# Autodesk Inventor assembly: Z Mount
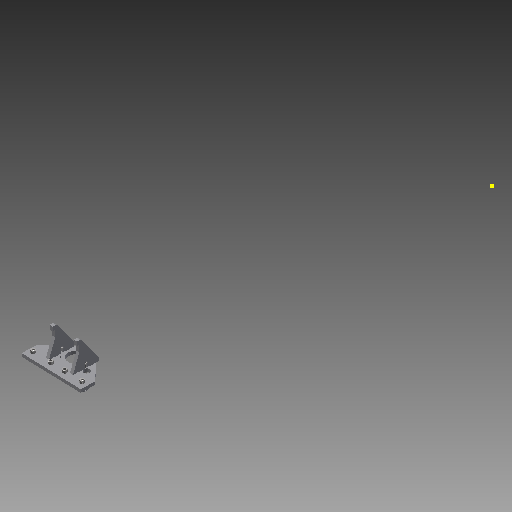
[picture p0: Inventor's stored thumbnail of the model, 512x512]
Saved by Autodesk Inventor 2017 (Build 210142000, 142)
## iProperties
Created: 2016-07-25
Part Number: Z Mount
Document SubType Name: Assembly
Designer: User
Author: User
## Documents named in this file (11)
- C:\All INVENTOR\SL-Inventor\SL-Beast 3D Printer\Z Mount.iam
- C:\All INVENTOR\SL-Inventor\SL-Beast 3D Printer\Rear Z Motor Mount.ipt
- C:\All INVENTOR\SL-Inventor\SL-Beast 3D Printer\Z Motor Mount Brace.ipt
- C:\All INVENTOR\SL-Inventor\SL-Beast 3D Printer\Z Motor Mount Brace_CPY.ipt
- C:\All INVENTOR\SL-Inventor\SL-Beast 3D Printer\en-US\ANSI B18.3.1M(6)\ANSI B18.3.1M - M3x0.5 x 16(1).ipt
- C:\All INVENTOR\SL-Inventor\SL-Beast 3D Printer\en-US\CSN EN 24 036\CSN EN 24 036 - M3.ipt
- C:\All INVENTOR\SL-Inventor\SL-Beast 3D Printer\en-US\ANSI B18.3.1M(6)\ANSI B18.3.1M - M5x0.8 x 12(1).ipt
- C:\All INVENTOR\SL-Inventor\SL-Beast 3D Printer\M5 Tee Nut-Generic_MIR1.ipt
- C:\All INVENTOR\SL-Inventor\SL-Beast 3D Printer\M5 Tee Nut-Generic_MIR1_CPY.ipt
- C:\All INVENTOR\SL-Inventor\SL-Beast 3D Printer\M5 Tee Nut-Generic_MIR1_CPY_CPY.ipt
- C:\All INVENTOR\SL-Inventor\SL-Beast 3D Printer\M5 Tee Nut-Generic_MIR1_CPY_CPY_CPY.ipt
## Components (15 placed, 10 different names)
1. Rear Z Motor Mount:1
2. Z Motor Mount Brace:1
3. Z Motor Mount Brace_CPY:1
4. Forged Socket Head Cap Screw - Metric M3x0.5 x 16:1
5. Forged Socket Head Cap Screw - Metric M3x0.5 x 16:2
6. CSN EN 24036 M3:1
7. CSN EN 24036 M3:2
8. Forged Socket Head Cap Screw - Metric M5x0.8 x 12:1
9. Forged Socket Head Cap Screw - Metric M5x0.8 x 12:2
10. Forged Socket Head Cap Screw - Metric M5x0.8 x 12:3
11. Forged Socket Head Cap Screw - Metric M5x0.8 x 12:4
12. M5 Tee Nut-Generic_MIR1:1
13. M5 Tee Nut-Generic_MIR1_CPY:1
14. M5 Tee Nut-Generic_MIR1_CPY_CPY:1
15. M5 Tee Nut-Generic_MIR1_CPY_CPY_CPY:1
## Relationships (24: Mate 14, Insert 6, Flush 4)
- [Mate]: Rear Z Motor Mount:1 ↔ Z Motor Mount Brace:1
- [Mate]: Rear Z Motor Mount:1 ↔ Z Motor Mount Brace:1
- [Mate]: Rear Z Motor Mount:1 ↔ Z Motor Mount Brace:1
- [Mate]: Rear Z Motor Mount:1 ↔ Z Motor Mount Brace_CPY:1
- [Flush]: Rear Z Motor Mount:1 ↔ Z Motor Mount Brace_CPY:1
- [Mate]: Rear Z Motor Mount:1 ↔ Z Motor Mount Brace_CPY:1
- [Insert]: Rear Z Motor Mount:1 ↔ Forged Socket Head Cap Screw - Metric M3x0.5 x 16:1
- [Insert]: Rear Z Motor Mount:1 ↔ Forged Socket Head Cap Screw - Metric M3x0.5 x 16:2
- [Mate]: Forged Socket Head Cap Screw - Metric M3x0.5 x 16:2 ↔ CSN EN 24036 M3:1
- [Mate]: Z Motor Mount Brace:1 ↔ CSN EN 24036 M3:1
- [Mate]: Forged Socket Head Cap Screw - Metric M3x0.5 x 16:1 ↔ CSN EN 24036 M3:2
- [Mate]: Z Motor Mount Brace_CPY:1 ↔ CSN EN 24036 M3:2
- [Insert]: Rear Z Motor Mount:1 ↔ Forged Socket Head Cap Screw - Metric M5x0.8 x 12:1
- [Insert]: Rear Z Motor Mount:1 ↔ Forged Socket Head Cap Screw - Metric M5x0.8 x 12:2
- [Insert]: Rear Z Motor Mount:1 ↔ Forged Socket Head Cap Screw - Metric M5x0.8 x 12:3
- [Insert]: Rear Z Motor Mount:1 ↔ Forged Socket Head Cap Screw - Metric M5x0.8 x 12:4
- [Mate]: Forged Socket Head Cap Screw - Metric M5x0.8 x 12:4 ↔ M5 Tee Nut-Generic_MIR1:1
- [Mate]: Forged Socket Head Cap Screw - Metric M5x0.8 x 12:3 ↔ M5 Tee Nut-Generic_MIR1_CPY:1
- [Mate]: Forged Socket Head Cap Screw - Metric M5x0.8 x 12:2 ↔ M5 Tee Nut-Generic_MIR1_CPY_CPY:1
- [Mate]: Forged Socket Head Cap Screw - Metric M5x0.8 x 12:1 ↔ M5 Tee Nut-Generic_MIR1_CPY_CPY_CPY:1
- [Flush]: M5 Tee Nut-Generic_MIR1_CPY_CPY:1 ↔ M5 Tee Nut-Generic_MIR1_CPY_CPY_CPY:1
- [Flush]: M5 Tee Nut-Generic_MIR1_CPY:1 ↔ M5 Tee Nut-Generic_MIR1_CPY_CPY:1
- [Flush]: M5 Tee Nut-Generic_MIR1:1 ↔ M5 Tee Nut-Generic_MIR1_CPY:1
- [Mate] (3 mm): Rear Z Motor Mount:1 ↔ M5 Tee Nut-Generic_MIR1_CPY_CPY_CPY:1
